# Autodesk Inventor assembly: SPE42 Base Paciente
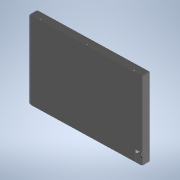
[picture p0: Inventor's stored thumbnail of the model, 180x180]
Saved by Autodesk Inventor 2021.2 (Build 252289000, 289)
## iProperties
Created: 2026-08-25
Part Number: SPE42 Base Paciente
Document SubType Name: Assembly
Designer: nelso
Author: nelso
## Documents named in this file (9)
- C:\Users\nelso\Desktop\Soporte-Paciente-Espinografia\Workspace\SPE42 Base Paciente.iam
- C:\Users\nelso\Desktop\Soporte-Paciente-Espinografia\Workspace\SP26V1 Base Chapa.ipt
- C:\Users\nelso\Desktop\Soporte-Paciente-Espinografia\Workspace\SP32V1 Refuerzo.ipt
- C:\Users\nelso\Desktop\Soporte-Paciente-Espinografia\Workspace\SP41V1 Cubre Base.ipt
- C:\Users\nelso\Desktop\Soporte-Paciente-Espinografia\Workspace\RFPLUS4PO300 Tuerca rem M4 cab red.ipt
- C:\Users\nelso\Desktop\Soporte-Paciente-Espinografia\Workspace\DIN7991M4X0.8L12C.ipt
- C:\Users\nelso\Desktop\Soporte-Paciente-Espinografia\Workspace\SP41V1 Goma Base.ipt
- C:\Users\nelso\Desktop\Soporte-Paciente-Espinografia\Workspace\SP40V1 Refuerzo pasador.ipt
- C:\Users\nelso\Desktop\Soporte-Paciente-Espinografia\Workspace\SKU1009783 -PasadorSCMetalurgica58mm.iam
## Components (19 placed, 8 different names)
1. SP26V1 Base Chapa:1
2. SP32V1 Refuerzo:1
3. SP40V1 Refuerzo pasador:1 — Mate:31, Flush:13, Mate:32, Mate:33
4. SP32V1 Refuerzo:3
5. SP41V1 Cubre Base:1
6. RFPLUS4PO300 Tuerca rem M4 cab red:1
7. RFPLUS4PO300 Tuerca rem M4 cab red:2
8. RFPLUS4PO300 Tuerca rem M4 cab red:3
9. RFPLUS4PO300 Tuerca rem M4 cab red:4
10. RFPLUS4PO300 Tuerca rem M4 cab red:5
11. RFPLUS4PO300 Tuerca rem M4 cab red:6
12. DIN7991M4X0.8L12C:1
13. DIN7991M4X0.8L12C:2
14. DIN7991M4X0.8L12C:3
15. DIN7991M4X0.8L12C:4
16. DIN7991M4X0.8L12C:5
17. DIN7991M4X0.8L12C:6
18. SP41V1 Goma Base:1
19. SKU1009783 -PasadorSCMetalurgica58mm:1 [sub-assembly] — Mate:31, Flush:13, Mate:32, Mate:33
## Relationships (43: Mate 30, Flush 13)
- [Mate]: SP26V1 Base Chapa:1 ↔ SP40V1 Refuerzo pasador:1
- [Mate]: SP26V1 Base Chapa:1 ↔ SP32V1 Refuerzo:3
- [Mate]: SP26V1 Base Chapa:1 ↔ SP32V1 Refuerzo:1
- [Mate]: SP26V1 Base Chapa:1 ↔ SP32V1 Refuerzo:3
- [Mate]: SP26V1 Base Chapa:1 ↔ SP40V1 Refuerzo pasador:1
- [Mate]: SP26V1 Base Chapa:1 ↔ SP32V1 Refuerzo:1
- [Flush]: SP26V1 Base Chapa:1 ↔ SP40V1 Refuerzo pasador:1
- [Flush]: SP26V1 Base Chapa:1 ↔ SP32V1 Refuerzo:1
- [Flush]: SP26V1 Base Chapa:1 ↔ SP32V1 Refuerzo:3
- [Flush]: SP26V1 Base Chapa:1 ↔ SP41V1 Cubre Base:1
- [Flush]: SP26V1 Base Chapa:1 ↔ SP41V1 Cubre Base:1
- [Flush] (2 mm): SP26V1 Base Chapa:1 ↔ SP41V1 Cubre Base:1
- [Mate]: SP26V1 Base Chapa:1 ↔ RFPLUS4PO300 Tuerca rem M4 cab red:6
- [Mate]: SP26V1 Base Chapa:1 ↔ RFPLUS4PO300 Tuerca rem M4 cab red:5
- [Mate]: SP26V1 Base Chapa:1 ↔ RFPLUS4PO300 Tuerca rem M4 cab red:4
- [Mate]: SP26V1 Base Chapa:1 ↔ RFPLUS4PO300 Tuerca rem M4 cab red:1
- [Mate]: SP26V1 Base Chapa:1 ↔ RFPLUS4PO300 Tuerca rem M4 cab red:2
- [Mate]: SP26V1 Base Chapa:1 ↔ RFPLUS4PO300 Tuerca rem M4 cab red:3
- [Mate]: SP26V1 Base Chapa:1 ↔ RFPLUS4PO300 Tuerca rem M4 cab red:1
- [Mate]: SP26V1 Base Chapa:1 ↔ RFPLUS4PO300 Tuerca rem M4 cab red:2
- [Mate]: SP26V1 Base Chapa:1 ↔ RFPLUS4PO300 Tuerca rem M4 cab red:3
- [Mate]: SP26V1 Base Chapa:1 ↔ RFPLUS4PO300 Tuerca rem M4 cab red:4
- [Mate]: SP26V1 Base Chapa:1 ↔ RFPLUS4PO300 Tuerca rem M4 cab red:5
- [Mate]: SP26V1 Base Chapa:1 ↔ RFPLUS4PO300 Tuerca rem M4 cab red:6
- [Mate]: SP26V1 Base Chapa:1 ↔ DIN7991M4X0.8L12C:1
- [Mate]: SP26V1 Base Chapa:1 ↔ DIN7991M4X0.8L12C:2
- [Mate]: SP26V1 Base Chapa:1 ↔ DIN7991M4X0.8L12C:3
- [Mate]: SP26V1 Base Chapa:1 ↔ DIN7991M4X0.8L12C:4
- [Mate]: SP26V1 Base Chapa:1 ↔ DIN7991M4X0.8L12C:5
- [Mate]: SP26V1 Base Chapa:1 ↔ DIN7991M4X0.8L12C:6
- [Flush]: SP26V1 Base Chapa:1 ↔ DIN7991M4X0.8L12C:3
- [Flush]: SP26V1 Base Chapa:1 ↔ DIN7991M4X0.8L12C:2
- [Flush]: SP26V1 Base Chapa:1 ↔ DIN7991M4X0.8L12C:1
- [Flush]: SP26V1 Base Chapa:1 ↔ DIN7991M4X0.8L12C:6
- [Flush]: SP26V1 Base Chapa:1 ↔ DIN7991M4X0.8L12C:5
- [Flush]: SP26V1 Base Chapa:1 ↔ DIN7991M4X0.8L12C:4
- [Mate]: SP26V1 Base Chapa:1 ↔ SP41V1 Goma Base:1
- [Mate]: SP26V1 Base Chapa:1 ↔ SP41V1 Goma Base:1
- [Mate]: SP26V1 Base Chapa:1 ↔ SP41V1 Goma Base:1
- Mate:31: SP40V1 Refuerzo pasador:1 ↔ SKU1009783 -PasadorSCMetalurgica58mm:1
- Flush:13: SP40V1 Refuerzo pasador:1 ↔ SKU1009783 -PasadorSCMetalurgica58mm:1
- Mate:32: SP40V1 Refuerzo pasador:1 ↔ SKU1009783 -PasadorSCMetalurgica58mm:1
- Mate:33: SP40V1 Refuerzo pasador:1 ↔ SKU1009783 -PasadorSCMetalurgica58mm:1
